# Autodesk Inventor assembly: plataforma inteira casa13
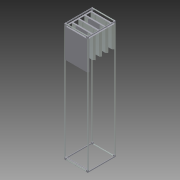
[picture p0: Inventor's stored thumbnail of the model, 180x180]
Saved by Autodesk Inventor 2013 (Build 170138000, 138)
## iProperties
Created: 2016-07-01
Part Number: plataforma inteira casa13
Document SubType Name: Assembly
Designer: New user
Mass: 4.89928e+06 g
Surface Area: 5.41775e+06 cm^2
Volume: 780204 cm^3
Density: 6.27948 g/cm^3
_SolveAssemblyDoc: Frame Generator Solve Assembly
_Version: 15.0.0
Author: New user
## Documents named in this file (9)
- W:\Mpm\Proj\inventor\plataforma inteira casa13.iam
- W:\Mpm\Proj\inventor\suporte longitudinal.ipt
- W:\Mpm\Proj\inventor\plataformafrt.iam
- W:\Mpm\Proj\inventor\corners40hicube.iam
- W:\Mpm\Proj\inventor\suporte transversal.ipt
- W:\Mpm\Proj\inventor\suporte alto.ipt
- W:\Mpm\Proj\inventor\drone1.iam
- W:\Mpm\Proj\inventor\Part6.ipt
- W:\Mpm\Proj\inventor\PLATAFORMA INTEIRA CASA\FRAME\FRAME0001.IAM
## Components (17 placed, 8 different names)
1. suporte longitudinal:1 — Flush:18, Flush:19, Mate:14
2. suporte longitudinal:2 — Mate:11, Flush:20, Mate:16
3. plataformafrt:1 [sub-assembly] — Flush:9, Mate:11, Mate:22, Flush:33
4. corners40hicube:1 [sub-assembly] — Flush:9, Mate:7, Mate:8, Mate:9, Mate:10, Flush:10, Mate:12, Mate:13, Flush:12, Flush:13, Flush:14, Flush:15, Flush:16, Flush:17, Flush:18, Flush:19, Mate:14, Mate:15, Flush:20, Mate:16, Flush:21, Flush:22, Mate:17, Flush:23, Flush:24, Mate:18, Flush:25, Flush:26, Flush:27, Flush:28, Mate:19, Flush:29, Flush:30, Mate:20, Flush:31, Flush:32, Mate:21, Mate:25
5. suporte longitudinal:3 — Mate:10, Flush:10, Flush:11, Flush:14, Mate:22, Flush:33
6. suporte longitudinal:4 — Mate:12, Flush:11, Flush:17, Mate:26
7. suporte transversal:1 — Mate:7, Mate:13, Flush:15, Flush:16, Flush:35
8. suporte transversal:2 — Mate:8, Flush:12, Flush:13
9. suporte transversal:3 — Mate:9, Mate:15, Flush:21, Flush:22
10. suporte transversal:4 — Mate:17, Flush:23, Flush:24
11. suporte alto:1 — Mate:18, Flush:25, Flush:26
12. suporte alto:2 — Flush:27, Flush:28, Mate:19
13. suporte alto:3 — Flush:29, Flush:30, Mate:20
14. suporte alto:4 — Flush:31, Flush:32, Mate:21
15. drone1:2 [sub-assembly]
16. Part6:1 — Flush:35
17. FRAME0001:1 [sub-assembly] — Mate:25, Mate:26
## Relationships (46: Flush 27, Mate 19)
- Flush:9: plataformafrt:1 ↔ corners40hicube:1
- Mate:7: corners40hicube:1 ↔ suporte transversal:1
- Mate:8: corners40hicube:1 ↔ suporte transversal:2
- Mate:9: corners40hicube:1 ↔ suporte transversal:3
- Mate:10: corners40hicube:1 ↔ suporte longitudinal:3
- Flush:10 (10 mm): corners40hicube:1 ↔ suporte longitudinal:3
- Mate:11: suporte longitudinal:2 ↔ plataformafrt:1
- Mate:12: corners40hicube:1 ↔ suporte longitudinal:4
- Flush:11: suporte longitudinal:3 ↔ suporte longitudinal:4
- Mate:13: corners40hicube:1 ↔ suporte transversal:1
- Flush:12: corners40hicube:1 ↔ suporte transversal:2
- Flush:13 (-10 mm): corners40hicube:1 ↔ suporte transversal:2
- Flush:14: corners40hicube:1 ↔ suporte longitudinal:3
- Flush:15 (-10 mm): corners40hicube:1 ↔ suporte transversal:1
- Flush:16: corners40hicube:1 ↔ suporte transversal:1
- Flush:17: corners40hicube:1 ↔ suporte longitudinal:4
- Flush:18 (-10 mm): suporte longitudinal:1 ↔ corners40hicube:1
- Flush:19 (-10 mm): suporte longitudinal:1 ↔ corners40hicube:1
- Mate:14: suporte longitudinal:1 ↔ corners40hicube:1
- Mate:15: corners40hicube:1 ↔ suporte transversal:3
- Flush:20: suporte longitudinal:2 ↔ corners40hicube:1
- Mate:16: suporte longitudinal:2 ↔ corners40hicube:1
- Flush:21: corners40hicube:1 ↔ suporte transversal:3
- Flush:22: corners40hicube:1 ↔ suporte transversal:3
- Mate:17: corners40hicube:1 ↔ suporte transversal:4
- Flush:23 (-10 mm): corners40hicube:1 ↔ suporte transversal:4
- Flush:24 (-10 mm): corners40hicube:1 ↔ suporte transversal:4
- Mate:18: corners40hicube:1 ↔ suporte alto:1
- Flush:25: corners40hicube:1 ↔ suporte alto:1
- Flush:26: corners40hicube:1 ↔ suporte alto:1
- Flush:27: corners40hicube:1 ↔ suporte alto:2
- Flush:28: corners40hicube:1 ↔ suporte alto:2
- Mate:19: corners40hicube:1 ↔ suporte alto:2
- Flush:29: corners40hicube:1 ↔ suporte alto:3
- Flush:30: corners40hicube:1 ↔ suporte alto:3
- Mate:20: corners40hicube:1 ↔ suporte alto:3
- Flush:31 (-10 mm): corners40hicube:1 ↔ suporte alto:4
- Flush:32 (-10 mm): corners40hicube:1 ↔ suporte alto:4
- Mate:21: corners40hicube:1 ↔ suporte alto:4
- Mate:22: plataformafrt:1 ↔ suporte longitudinal:3
- Flush:33: plataformafrt:1 ↔ suporte longitudinal:3
- [Mate] (10 mm): plataformafrt:1 ↔ drone1:2
- Flush:35: suporte transversal:1 ↔ Part6:1
- [Flush] (30 mm): suporte longitudinal:3 ↔ FRAME0001:1
- Mate:25: corners40hicube:1 ↔ FRAME0001:1
- Mate:26: suporte longitudinal:4 ↔ FRAME0001:1
